# Autodesk Inventor assembly: Pakiet_blaczek_d
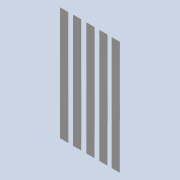
[picture p0: Inventor's stored thumbnail of the model, 180x180]
Saved by Autodesk Inventor 2021.3 (Build 253353000, 353)
## iProperties
Created: 2023-05-23
Part Number: Pakiet_blaczek_d
Document SubType Name: Assembly
Designer: User
Author: User
## Documents named in this file (2)
- E:\Inventor\Projekty\Modele Robotyzacja Procesów\Pakiet_blaczek_d.iam
- E:\Inventor\Projekty\Modele Robotyzacja Procesów\tasiemka_do_zgrzewania_2.ipt
## Components (5 placed, 1 different names)
1. tasiemka_do_zgrzewania_2:1 — Równoległe:12, Równoległe:13, Zestawiające:18, Zestawiające:19
2. tasiemka_do_zgrzewania_2:2 — Równoległe:13, Równoległe:14, Zestawiające:19, Zestawiające:20
3. tasiemka_do_zgrzewania_2:3 — Równoległe:14, Równoległe:15, Zestawiające:20
4. tasiemka_do_zgrzewania_2:4 — Równoległe:15
5. tasiemka_do_zgrzewania_2:5 — Równoległe:12, Zestawiające:18
## Relationships (7: Flush 4, Mate 3)
- Równoległe:12 [Flush]: tasiemka_do_zgrzewania_2:1 ↔ tasiemka_do_zgrzewania_2:5
- Równoległe:13 [Flush]: tasiemka_do_zgrzewania_2:1 ↔ tasiemka_do_zgrzewania_2:2
- Równoległe:14 [Flush]: tasiemka_do_zgrzewania_2:2 ↔ tasiemka_do_zgrzewania_2:3
- Równoległe:15 [Flush]: tasiemka_do_zgrzewania_2:3 ↔ tasiemka_do_zgrzewania_2:4
- Zestawiające:18 [Mate] (44 mm): tasiemka_do_zgrzewania_2:1 ↔ tasiemka_do_zgrzewania_2:5
- Zestawiające:19 [Mate] (44 mm): tasiemka_do_zgrzewania_2:1 ↔ tasiemka_do_zgrzewania_2:2
- Zestawiające:20 [Mate] (44 mm): tasiemka_do_zgrzewania_2:2 ↔ tasiemka_do_zgrzewania_2:3
